# Autodesk Inventor assembly: complete_assembly
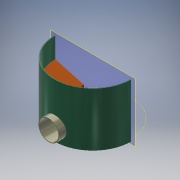
[picture p0: Inventor's stored thumbnail of the model, 180x180]
Saved by Autodesk Inventor 2019 (Build 230136000, 136)
## iProperties
Created: 2019-05-05
Part Number: complete_assembly
Document SubType Name: Assembly
Designer: assman
Author: assman
## Documents named in this file (6)
- D:\Inventor\Projects\CatFeeder\Case\version7\complete_assembly.iam
- D:\Inventor\Projects\CatFeeder\Case\version7\base.ipt
- D:\Inventor\Projects\CatFeeder\Case\version7\case.ipt
- D:\Inventor\Projects\CatFeeder\Case\version7\cap.ipt
- D:\Inventor\Projects\CatFeeder\Case\version7\inner_cone.ipt
- D:\Inventor\Projects\CatFeeder\Case\version7\auger_assembly.iam
## Components (5 placed, 5 different names)
1. base:1
2. case:1 — Rigid:1
3. cap:1
4. inner_cone:1 — Cylindrical:1
5. auger_assembly:1 [sub-assembly] — Rigid:1, Cylindrical:1
## Relationships (2: WeldJoint 1, CylindricalJoint 1)
- Rigid:1 [WeldJoint]: case:1 ↔ auger_assembly:1
- Cylindrical:1: inner_cone:1 ↔ auger_assembly:1
